# Autodesk Inventor assembly: 000 Ensamblaje_3d_Welding_Tooling - BASIC
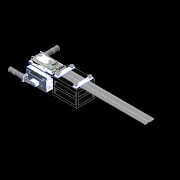
[picture p0: Inventor's stored thumbnail of the model, 180x180]
Saved by Autodesk Inventor 2018.3 (Build 223284000, 284)
## iProperties
Created: 2026-01-13
Part Number: 000 Ensamblaje_3d_Welding_Tooling - BASIC
Document SubType Name: Assembly
Designer: aca6
Mass: 2650.67 g
Surface Area: 3394.3 cm^2
Volume: 1053.59 cm^3
Density: 2.51584 g/cm^3
Manufacturer-1: {"Name": "Embention Sistemas Inteligentes S.A.", "PartNumber": "3d_Welding_Tooling - BASIC", "Link": ""}
Manufacturer-2: {"Name": "", "PartNumber": "", "Link": ""}
Manufacturer-3: {"Name": "", "PartNumber": "", "Link": ""}
Manufacturer-4: {"Name": "", "PartNumber": "", "Link": ""}
Manufacturer-5: {"Name": "", "PartNumber": "", "Link": ""}
Provider-1: {"Name": "", "PartNumber": "", "Link": ""}
Provider-2: {"Name": "", "PartNumber": "", "Link": ""}
Provider-3: {"Name": "", "PartNumber": "", "Link": ""}
Provider-4: {"Name": "", "PartNumber": "", "Link": ""}
Provider-5: {"Name": "", "PartNumber": "", "Link": ""}
Author: aca6
## Documents named in this file (29)
- C:\Users\aca6\git\LM\items\hw_LM\variants\items\Welding Tooling\3d\000 Ensamblaje_3d_Welding_Tooling - BASIC.iam
- C:\Users\aca6\git\LM\items\hw_LM\variants\items\Welding Tooling\3d\3d_Welding_Tooling - Adapter.ipt
- C:\Users\aca6\git\LM\items\hw_LM\variants\items\Welding Tooling\3d\3d_Welding_Tooling - Welding Placement.ipt
- C:\Users\aca6\git\LM\items\hw_LM\variants\items\Welding Tooling\3d\3d_Welding_Tooling -  Guide Pin.ipt
- C:\Users\aca6\git\LM\items\hw_LM\variants\items\Welding Tooling\3d\3d_Welding_Tooling - Wire.ipt
- C:\Users\aca6\git\LM\items\hw_LM\variants\items\Welding Tooling\3d\3d_Welding_Tooling - Bot Wire.ipt
- C:\Users\aca6\git\LM\items\hw_LM\variants\items\Welding Tooling\3d\3d_Welding_Tooling - Top Adapter.ipt
- C:\Users\aca6\git\LM\items\hw_LM\variants\items\Welding Tooling\3d\3d_Welding_Tooling - Moving base.ipt
- C:\Users\aca6\git\LM\items\hw_LM\variants\items\Welding Tooling\3d\3d_Welding_Tooling - Fixed base.ipt
- C:\Users\aca6\git\LM\items\hw_LM\variants\items\Welding Tooling\3d\3d_Welding_Tooling - Acetal Stick.ipt
- C:\Users\aca6\git\LM\items\hw_LM\variants\items\Welding Tooling\3d\3d_Welding_Tooling -  4x14 Guide Pin.ipt
- C:\Users\aca6\git\LM\items\hw_LM\variants\items\Welding Tooling\3d\3d_Welding_Tooling - Upper fixed base.ipt
- C:\Users\aca6\git\LM\items\hw_LM\variants\items\Welding Tooling\3d\3d_Welding_Tooling - Upper moving base.ipt
- C:\Users\aca6\git\LM\items\_accesories\Tornilleria\Tornillos\3d_DIN 7991\3d\A4 Black Inox\DIN 7991 - M3x14 Black INOX.ipt
- C:\Users\aca6\git\LM\items\_accesories\Tornilleria\Tornillos\3d_DIN 7991\3d\A4 Black Inox\DIN 7991 - M3x12 Black INOX.ipt
- C:\Users\aca6\git\LM\items\hw_LM\variants\items\Welding Tooling\3d\3d_Welding_Tooling -  Micrometer.ipt
- C:\Users\aca6\git\LM\items\hw_LM\variants\items\Welding Tooling\3d\3d_Welding_Tooling -  Micrometer Nut.ipt
- C:\Users\aca6\git\LM\items\hw_LM\variants\items\Welding Tooling\3d\3d_Welding_Tooling - Fixed Block.ipt
- C:\Users\aca6\git\LM\items\hw_LM\variants\items\Welding Tooling\3d\3d_Welding_Tooling -  Tab.ipt
- C:\Users\aca6\git\LM\items\hw_LM\variants\items\Welding Tooling\3d\3d_Welding_Tooling -  Moving Block.ipt
- C:\Users\aca6\git\LM\items\_accesories\Tornilleria\Tornillos\3d_Accu Group\3d\Prisionero nylon M4x7 REF SSN-M4-7.ipt
- C:\Users\aca6\git\LM\items\_accesories\Tornilleria\Tornillos\3d_DIN 912\3d\A4 Inox\DIN 912 - M3 x 0,5 x 8 -  INOX.ipt
- C:\Users\aca6\git\LM\items\_accesories\Tornilleria\Tornillos\3d_DIN 912\3d\A4 Inox\DIN 912 - M3 x 0,5 x 30 -  INOX.ipt
- C:\Users\aca6\git\LM\items\_accesories\Tornilleria\Tornillos\3d_DIN 912\3d\A4 Inox\DIN 912 - M3 x 0,5 x 10 -  INOX.ipt
- C:\Users\aca6\git\LM\items\_accesories\Tornilleria\Insertos\3d_Genéricos\3d\Inserto roscado M4x5.6x7.95.ipt
- C:\Users\aca6\git\LM\items\hw_LM\variants\items\Welding Tooling\3d\Knurled Screw_ Stainless Steel DIN 464-M4-10-A4.ipt
- C:\Users\aca6\git\LM\items\3d_LM\variants\BASIC\dummy\3d_LM - BASIC - welding tooling_dummy.ipt
- C:\Users\aca6\git\LM\items\3d_LM\3d\3d_LM - Bottom Wire - Phantom.ipt
- C:\Users\aca6\git\LM\items\3d_LM\3d\3d_LM - Top Wire - Phantom.ipt
## Components (69 placed, 28 different names)
1. 3d_Welding_Tooling - Adapter:1 — Flush:3, Mate:12, Mate:13, Mate:14, Mate:15, Mate:16, Mate:22, Mate:23, Mate:24, Flush:14, Mate:89, Mate:107, Flush:28, Flush:29, Mate:108, Mate:109, Mate:110, Mate:111, Tangent:5, Tangent:6, Tangent:7, Tangent:8, Flush:120
2. 3d_Welding_Tooling - Welding Placement:1 — Flush:3, Mate:89, Flush:120, Mate:126, Mate:127, Mate:128, Mate:129, Mate:130, Mate:131, Mate:136, Mate:137, Mate:204, Mate:205, Mate:206, Mate:207, Mate:208, Flush:141, Flush:142, Flush:143
3. 3d_Welding_Tooling -  Guide Pin:1 — Mate:12, Mate:16, Mate:23, Mate:50, Mate:238
4. 3d_Welding_Tooling -  Guide Pin:2 — Mate:13, Mate:15, Mate:22, Mate:49, Mate:239
5. 3d_Welding_Tooling -  Guide Pin:3 — Mate:14, Mate:24
6. 3d_Welding_Tooling - Top Adapter:1 — Flush:14, Mate:49, Mate:50, Mate:240
7. 3d_Welding_Tooling - Moving base:1 — Mate:58, Flush:18, Mate:59, Mate:60, Mate:94, Mate:95, Mate:96, Flush:123, Mate:173, Flush:140
8. 3d_Welding_Tooling - Fixed base:1 — Mate:58, Flush:18, Flush:19, Mate:61, Mate:62, Flush:20, Flush:123, Mate:163, Mate:165, Flush:124, Flush:125, Mate:168, Flush:129, Flush:130, Mate:178, Flush:135, Mate:179, Flush:136
9. 3d_Welding_Tooling - Acetal Stick:1 — Mate:59, Mate:60, Flush:19
10. 3d_Welding_Tooling - Acetal Stick:2 — Mate:61, Mate:62, Flush:20
11. 3d_Welding_Tooling -  4x14 Guide Pin:1 — Mate:128, Mate:129
12. 3d_Welding_Tooling -  4x14 Guide Pin:2 — Mate:126, Mate:127
13. 3d_Welding_Tooling - Upper fixed base:1 — Mate:94, Mate:95, Mate:96, Mate:97, Mate:98, Mate:99, Mate:100, Flush:26, Flush:27, Mate:101, Mate:103, Mate:104, Mate:105, Mate:106, Tangent:1, Tangent:2, Tangent:3, Tangent:4, Mate:158, Flush:121, Flush:122, Mate:162, Mate:164, Flush:126, Flush:127, Flush:128, Mate:180, Flush:137, Mate:181, Flush:138
14. 3d_Welding_Tooling - Acetal Stick:3 — Mate:97, Mate:98, Flush:27
15. 3d_Welding_Tooling - Acetal Stick:4 — Mate:99, Mate:100, Flush:26, Mate:102
16. 3d_Welding_Tooling - Upper moving base:1 — Mate:101, Mate:102, Mate:107, Flush:28, Flush:29, Mate:160, Flush:122, Mate:174, Mate:175, Mate:176, Mate:177, Flush:131, Flush:132, Flush:133, Flush:134, Flush:139
17. DIN 7991 - M3x14 Black INOX:1 — Mate:105, Tangent:3
18. DIN 7991 - M3x14 Black INOX:2 — Mate:106, Tangent:2
19. DIN 7991 - M3x14 Black INOX:3 — Mate:103, Tangent:4
20. DIN 7991 - M3x14 Black INOX:4 — Mate:104, Tangent:1
21. DIN 7991 - M3x12 Black INOX:1 — Mate:109, Tangent:8
22. DIN 7991 - M3x12 Black INOX:2 — Mate:111, Tangent:6
23. DIN 7991 - M3x12 Black INOX:3 — Mate:110, Tangent:5
24. DIN 7991 - M3x12 Black INOX:4 — Mate:108, Tangent:7
25. 3d_Welding_Tooling -  Micrometer Nut:1 — Mate:171, Mate:172
26. 3d_Welding_Tooling -  Tab:1 — Mate:130, Mate:131, Mate:217, Mate:223
27. 3d_Welding_Tooling -  Tab:2 — Mate:136, Mate:137, Mate:219, Mate:221
28. 3d_Welding_Tooling -  Micrometer:2 — Mate:187
29. 3d_Welding_Tooling -  Micrometer Nut:2
30. 3d_Welding_Tooling - Fixed Block:2 — Mate:158, Flush:121, Flush:128, Mate:196, Mate:197, Mate:198, Mate:199
31. 3d_Welding_Tooling -  Moving Block:1 — Mate:160, Mate:184, Mate:185, Mate:187, Flush:139, Mate:192, Mate:193, Mate:194, Mate:195
32. Prisionero nylon M4x7 REF SSN-M4-7:1 — Mate:162, Flush:126
33. Prisionero nylon M4x7 REF SSN-M4-7:2 — Mate:163, Flush:125
34. Prisionero nylon M4x7 REF SSN-M4-7:3 — Mate:165, Flush:124
35. Prisionero nylon M4x7 REF SSN-M4-7:4 — Mate:164, Flush:127
36. 3d_Welding_Tooling - Fixed Block:3 — Mate:168, Flush:129, Flush:130, Mate:169, Mate:170, Mate:172, Mate:200, Mate:201, Mate:202, Mate:203
37. 3d_Welding_Tooling -  Micrometer:3 — Mate:169, Mate:170, Mate:171, Mate:186
38. 3d_Welding_Tooling -  Moving Block:2 — Mate:173, Mate:182, Mate:183, Mate:186, Flush:140, Mate:188, Mate:189, Mate:190, Mate:191
39. Prisionero nylon M4x7 REF SSN-M4-7:5 — Mate:174, Flush:132
40. Prisionero nylon M4x7 REF SSN-M4-7:6 — Mate:177, Flush:131
41. Prisionero nylon M4x7 REF SSN-M4-7:7 — Mate:176, Flush:133
42. Prisionero nylon M4x7 REF SSN-M4-7:8 — Mate:175, Flush:134
43. Prisionero nylon M4x7 REF SSN-M4-7:9 — Mate:178, Flush:135
44. Prisionero nylon M4x7 REF SSN-M4-7:10 — Mate:179, Flush:136
45. Prisionero nylon M4x7 REF SSN-M4-7:11 — Mate:180, Flush:137
46. Prisionero nylon M4x7 REF SSN-M4-7:12 — Mate:181, Flush:138
47. DIN 912 - M3 x 0,5 x 8 -  INOX:1 — Mate:184, Mate:185
48. DIN 912 - M3 x 0,5 x 8 -  INOX:2 — Mate:182, Mate:183
49. DIN 912 - M3 x 0,5 x 30 -  INOX:4 — Mate:189, Mate:191
50. DIN 912 - M3 x 0,5 x 30 -  INOX:3 — Mate:188, Mate:190
51. DIN 912 - M3 x 0,5 x 30 -  INOX:1 — Mate:192, Mate:195
52. DIN 912 - M3 x 0,5 x 30 -  INOX:2 — Mate:193, Mate:194
53. DIN 912 - M3 x 0,5 x 10 -  INOX:1 — Mate:197, Mate:198
54. DIN 912 - M3 x 0,5 x 10 -  INOX:2 — Mate:196, Mate:199
55. DIN 912 - M3 x 0,5 x 10 -  INOX:3 — Mate:201, Mate:202
56. DIN 912 - M3 x 0,5 x 10 -  INOX:4 — Mate:200, Mate:203
57. Inserto roscado M4x5.6x7.95:1 — Mate:204, Mate:205, Mate:216
58. Inserto roscado M4x5.6x7.95:2 — Mate:207, Flush:143, Mate:218
59. Inserto roscado M4x5.6x7.95:3 — Mate:208, Flush:142, Mate:220
60. Inserto roscado M4x5.6x7.95:4 — Mate:206, Flush:141, Mate:222
61. Knurled Screw_ Stainless Steel DIN 464-M4-10-A4:1 — Mate:216, Mate:217
62. Knurled Screw_ Stainless Steel DIN 464-M4-10-A4:2 — Mate:222, Mate:223
63. Knurled Screw_ Stainless Steel DIN 464-M4-10-A4:3 — Mate:220, Mate:221
64. Knurled Screw_ Stainless Steel DIN 464-M4-10-A4:4 — Mate:218, Mate:219
65. 3d_LM - Top Wire - Phantom:1 — Mate:244, Mate:245, Mate:246, Mate:250, Mate:251, Mate:252
66. 3d_LM - Bottom Wire - Phantom:1 — Mate:241, Mate:242, Mate:243, Mate:247, Mate:248, Mate:249
67. 3d_LM - BASIC - welding tooling_dummy:1 — Mate:238, Mate:239, Mate:240, Mate:247, Mate:248, Mate:249, Mate:250, Mate:251, Mate:252
68. 3d_Welding_Tooling - Wire:1 — Mate:244, Mate:245, Mate:246
69. 3d_Welding_Tooling - Bot Wire:1 — Mate:241, Mate:242, Mate:243
## Relationships (157: Mate 116, Flush 33, Tangent 8)
- Flush:3 (-60 mm): 3d_Welding_Tooling - Adapter:1 ↔ 3d_Welding_Tooling - Welding Placement:1
- Mate:12: 3d_Welding_Tooling - Adapter:1 ↔ 3d_Welding_Tooling -  Guide Pin:1
- Mate:13: 3d_Welding_Tooling - Adapter:1 ↔ 3d_Welding_Tooling -  Guide Pin:2
- Mate:14: 3d_Welding_Tooling - Adapter:1 ↔ 3d_Welding_Tooling -  Guide Pin:3
- Mate:15: 3d_Welding_Tooling - Adapter:1 ↔ 3d_Welding_Tooling -  Guide Pin:2
- Mate:16: 3d_Welding_Tooling - Adapter:1 ↔ 3d_Welding_Tooling -  Guide Pin:1
- Mate:22: 3d_Welding_Tooling - Adapter:1 ↔ 3d_Welding_Tooling -  Guide Pin:2
- Mate:23: 3d_Welding_Tooling - Adapter:1 ↔ 3d_Welding_Tooling -  Guide Pin:1
- Mate:24: 3d_Welding_Tooling - Adapter:1 ↔ 3d_Welding_Tooling -  Guide Pin:3
- Flush:14: 3d_Welding_Tooling - Adapter:1 ↔ 3d_Welding_Tooling - Top Adapter:1
- Mate:49: 3d_Welding_Tooling -  Guide Pin:2 ↔ 3d_Welding_Tooling - Top Adapter:1
- Mate:50: 3d_Welding_Tooling -  Guide Pin:1 ↔ 3d_Welding_Tooling - Top Adapter:1
- Mate:58: 3d_Welding_Tooling - Moving base:1 ↔ 3d_Welding_Tooling - Fixed base:1
- Flush:18: 3d_Welding_Tooling - Moving base:1 ↔ 3d_Welding_Tooling - Fixed base:1
- Mate:59: 3d_Welding_Tooling - Moving base:1 ↔ 3d_Welding_Tooling - Acetal Stick:1
- Mate:60: 3d_Welding_Tooling - Moving base:1 ↔ 3d_Welding_Tooling - Acetal Stick:1
- Mate:61: 3d_Welding_Tooling - Fixed base:1 ↔ 3d_Welding_Tooling - Acetal Stick:2
- Mate:62: 3d_Welding_Tooling - Fixed base:1 ↔ 3d_Welding_Tooling - Acetal Stick:2
- Flush:19: 3d_Welding_Tooling - Fixed base:1 ↔ 3d_Welding_Tooling - Acetal Stick:1
- Flush:20: 3d_Welding_Tooling - Fixed base:1 ↔ 3d_Welding_Tooling - Acetal Stick:2
- Mate:89 (3 mm): 3d_Welding_Tooling - Adapter:1 ↔ 3d_Welding_Tooling - Welding Placement:1
- Mate:94: 3d_Welding_Tooling - Moving base:1 ↔ 3d_Welding_Tooling - Upper fixed base:1
- Mate:95: 3d_Welding_Tooling - Moving base:1 ↔ 3d_Welding_Tooling - Upper fixed base:1
- Mate:96: 3d_Welding_Tooling - Moving base:1 ↔ 3d_Welding_Tooling - Upper fixed base:1
- Mate:97: 3d_Welding_Tooling - Upper fixed base:1 ↔ 3d_Welding_Tooling - Acetal Stick:3
- Mate:98: 3d_Welding_Tooling - Upper fixed base:1 ↔ 3d_Welding_Tooling - Acetal Stick:3
- Mate:99: 3d_Welding_Tooling - Upper fixed base:1 ↔ 3d_Welding_Tooling - Acetal Stick:4
- Mate:100: 3d_Welding_Tooling - Upper fixed base:1 ↔ 3d_Welding_Tooling - Acetal Stick:4
- Flush:26: 3d_Welding_Tooling - Upper fixed base:1 ↔ 3d_Welding_Tooling - Acetal Stick:4
- Flush:27: 3d_Welding_Tooling - Upper fixed base:1 ↔ 3d_Welding_Tooling - Acetal Stick:3
- Mate:101: 3d_Welding_Tooling - Upper fixed base:1 ↔ 3d_Welding_Tooling - Upper moving base:1
- Mate:102: 3d_Welding_Tooling - Acetal Stick:4 ↔ 3d_Welding_Tooling - Upper moving base:1
- Mate:103: 3d_Welding_Tooling - Upper fixed base:1 ↔ DIN 7991 - M3x14 Black INOX:3
- Mate:104: 3d_Welding_Tooling - Upper fixed base:1 ↔ DIN 7991 - M3x14 Black INOX:4
- Mate:105: 3d_Welding_Tooling - Upper fixed base:1 ↔ DIN 7991 - M3x14 Black INOX:1
- Mate:106: 3d_Welding_Tooling - Upper fixed base:1 ↔ DIN 7991 - M3x14 Black INOX:2
- Tangent:1: 3d_Welding_Tooling - Upper fixed base:1 ↔ DIN 7991 - M3x14 Black INOX:4
- Tangent:2: 3d_Welding_Tooling - Upper fixed base:1 ↔ DIN 7991 - M3x14 Black INOX:2
- Tangent:3: 3d_Welding_Tooling - Upper fixed base:1 ↔ DIN 7991 - M3x14 Black INOX:1
- Tangent:4: 3d_Welding_Tooling - Upper fixed base:1 ↔ DIN 7991 - M3x14 Black INOX:3
- Mate:107: 3d_Welding_Tooling - Adapter:1 ↔ 3d_Welding_Tooling - Upper moving base:1
- Flush:28 (18.75 mm): 3d_Welding_Tooling - Adapter:1 ↔ 3d_Welding_Tooling - Upper moving base:1
- Flush:29 (-9.684 mm): 3d_Welding_Tooling - Adapter:1 ↔ 3d_Welding_Tooling - Upper moving base:1
- Mate:108: 3d_Welding_Tooling - Adapter:1 ↔ DIN 7991 - M3x12 Black INOX:4
- Mate:109: 3d_Welding_Tooling - Adapter:1 ↔ DIN 7991 - M3x12 Black INOX:1
- Mate:110: 3d_Welding_Tooling - Adapter:1 ↔ DIN 7991 - M3x12 Black INOX:3
- Mate:111: 3d_Welding_Tooling - Adapter:1 ↔ DIN 7991 - M3x12 Black INOX:2
- Tangent:5: 3d_Welding_Tooling - Adapter:1 ↔ DIN 7991 - M3x12 Black INOX:3
- Tangent:6: 3d_Welding_Tooling - Adapter:1 ↔ DIN 7991 - M3x12 Black INOX:2
- Tangent:7: 3d_Welding_Tooling - Adapter:1 ↔ DIN 7991 - M3x12 Black INOX:4
- Tangent:8: 3d_Welding_Tooling - Adapter:1 ↔ DIN 7991 - M3x12 Black INOX:1
- Flush:120 (-13.75 mm): 3d_Welding_Tooling - Adapter:1 ↔ 3d_Welding_Tooling - Welding Placement:1
- Mate:126: 3d_Welding_Tooling - Welding Placement:1 ↔ 3d_Welding_Tooling -  4x14 Guide Pin:2
- Mate:127: 3d_Welding_Tooling - Welding Placement:1 ↔ 3d_Welding_Tooling -  4x14 Guide Pin:2
- Mate:128: 3d_Welding_Tooling - Welding Placement:1 ↔ 3d_Welding_Tooling -  4x14 Guide Pin:1
- Mate:129: 3d_Welding_Tooling - Welding Placement:1 ↔ 3d_Welding_Tooling -  4x14 Guide Pin:1
- Mate:130 (2.5 mm): 3d_Welding_Tooling - Welding Placement:1 ↔ 3d_Welding_Tooling -  Tab:1
- Mate:131: 3d_Welding_Tooling - Welding Placement:1 ↔ 3d_Welding_Tooling -  Tab:1
- Mate:136: 3d_Welding_Tooling - Welding Placement:1 ↔ 3d_Welding_Tooling -  Tab:2
- Mate:137 (2.5 mm): 3d_Welding_Tooling - Welding Placement:1 ↔ 3d_Welding_Tooling -  Tab:2
- [Mate]: 3d_Welding_Tooling -  Micrometer:2 ↔ 3d_Welding_Tooling - Fixed Block:2
- [Mate]: 3d_Welding_Tooling -  Micrometer:2 ↔ 3d_Welding_Tooling - Fixed Block:2
- [Mate]: 3d_Welding_Tooling -  Micrometer:2 ↔ 3d_Welding_Tooling -  Micrometer Nut:2
- [Mate]: 3d_Welding_Tooling -  Micrometer Nut:2 ↔ 3d_Welding_Tooling - Fixed Block:2
- Mate:158: 3d_Welding_Tooling - Upper fixed base:1 ↔ 3d_Welding_Tooling - Fixed Block:2
- Flush:121: 3d_Welding_Tooling - Upper fixed base:1 ↔ 3d_Welding_Tooling - Fixed Block:2
- Mate:160: 3d_Welding_Tooling - Upper moving base:1 ↔ 3d_Welding_Tooling -  Moving Block:1
- Flush:122: 3d_Welding_Tooling - Upper fixed base:1 ↔ 3d_Welding_Tooling - Upper moving base:1
- Flush:123: 3d_Welding_Tooling - Moving base:1 ↔ 3d_Welding_Tooling - Fixed base:1
- Mate:162: 3d_Welding_Tooling - Upper fixed base:1 ↔ Prisionero nylon M4x7 REF SSN-M4-7:1
- Mate:163: 3d_Welding_Tooling - Fixed base:1 ↔ Prisionero nylon M4x7 REF SSN-M4-7:2
- Mate:164: 3d_Welding_Tooling - Upper fixed base:1 ↔ Prisionero nylon M4x7 REF SSN-M4-7:4
- Mate:165: 3d_Welding_Tooling - Fixed base:1 ↔ Prisionero nylon M4x7 REF SSN-M4-7:3
- Flush:124: 3d_Welding_Tooling - Fixed base:1 ↔ Prisionero nylon M4x7 REF SSN-M4-7:3
- Flush:125: 3d_Welding_Tooling - Fixed base:1 ↔ Prisionero nylon M4x7 REF SSN-M4-7:2
- Flush:126: 3d_Welding_Tooling - Upper fixed base:1 ↔ Prisionero nylon M4x7 REF SSN-M4-7:1
- Flush:127: 3d_Welding_Tooling - Upper fixed base:1 ↔ Prisionero nylon M4x7 REF SSN-M4-7:4
- Flush:128: 3d_Welding_Tooling - Upper fixed base:1 ↔ 3d_Welding_Tooling - Fixed Block:2
- Mate:168: 3d_Welding_Tooling - Fixed base:1 ↔ 3d_Welding_Tooling - Fixed Block:3
- Flush:129: 3d_Welding_Tooling - Fixed base:1 ↔ 3d_Welding_Tooling - Fixed Block:3
- Flush:130: 3d_Welding_Tooling - Fixed base:1 ↔ 3d_Welding_Tooling - Fixed Block:3
- Mate:169: 3d_Welding_Tooling - Fixed Block:3 ↔ 3d_Welding_Tooling -  Micrometer:3
- Mate:170: 3d_Welding_Tooling - Fixed Block:3 ↔ 3d_Welding_Tooling -  Micrometer:3
- Mate:171: 3d_Welding_Tooling -  Micrometer Nut:1 ↔ 3d_Welding_Tooling -  Micrometer:3
- Mate:172: 3d_Welding_Tooling -  Micrometer Nut:1 ↔ 3d_Welding_Tooling - Fixed Block:3
- Mate:173: 3d_Welding_Tooling - Moving base:1 ↔ 3d_Welding_Tooling -  Moving Block:2
- Mate:174: 3d_Welding_Tooling - Upper moving base:1 ↔ Prisionero nylon M4x7 REF SSN-M4-7:5
- Mate:175: 3d_Welding_Tooling - Upper moving base:1 ↔ Prisionero nylon M4x7 REF SSN-M4-7:8
- Mate:176: 3d_Welding_Tooling - Upper moving base:1 ↔ Prisionero nylon M4x7 REF SSN-M4-7:7
- Mate:177: 3d_Welding_Tooling - Upper moving base:1 ↔ Prisionero nylon M4x7 REF SSN-M4-7:6
- Flush:131: 3d_Welding_Tooling - Upper moving base:1 ↔ Prisionero nylon M4x7 REF SSN-M4-7:6
- Flush:132: 3d_Welding_Tooling - Upper moving base:1 ↔ Prisionero nylon M4x7 REF SSN-M4-7:5
- Flush:133: 3d_Welding_Tooling - Upper moving base:1 ↔ Prisionero nylon M4x7 REF SSN-M4-7:7
- Flush:134: 3d_Welding_Tooling - Upper moving base:1 ↔ Prisionero nylon M4x7 REF SSN-M4-7:8
- Mate:178: 3d_Welding_Tooling - Fixed base:1 ↔ Prisionero nylon M4x7 REF SSN-M4-7:9
- Flush:135: 3d_Welding_Tooling - Fixed base:1 ↔ Prisionero nylon M4x7 REF SSN-M4-7:9
- Mate:179: 3d_Welding_Tooling - Fixed base:1 ↔ Prisionero nylon M4x7 REF SSN-M4-7:10
- Flush:136: 3d_Welding_Tooling - Fixed base:1 ↔ Prisionero nylon M4x7 REF SSN-M4-7:10
- Mate:180: 3d_Welding_Tooling - Upper fixed base:1 ↔ Prisionero nylon M4x7 REF SSN-M4-7:11
- Flush:137: 3d_Welding_Tooling - Upper fixed base:1 ↔ Prisionero nylon M4x7 REF SSN-M4-7:11
- Mate:181: 3d_Welding_Tooling - Upper fixed base:1 ↔ Prisionero nylon M4x7 REF SSN-M4-7:12
- Flush:138: 3d_Welding_Tooling - Upper fixed base:1 ↔ Prisionero nylon M4x7 REF SSN-M4-7:12
- Mate:182: 3d_Welding_Tooling -  Moving Block:2 ↔ DIN 912 - M3 x 0,5 x 8 -  INOX:2
- Mate:183: 3d_Welding_Tooling -  Moving Block:2 ↔ DIN 912 - M3 x 0,5 x 8 -  INOX:2
- Mate:184: 3d_Welding_Tooling -  Moving Block:1 ↔ DIN 912 - M3 x 0,5 x 8 -  INOX:1
- Mate:185: 3d_Welding_Tooling -  Moving Block:1 ↔ DIN 912 - M3 x 0,5 x 8 -  INOX:1
- Mate:186: 3d_Welding_Tooling -  Micrometer:3 ↔ 3d_Welding_Tooling -  Moving Block:2
- Mate:187: 3d_Welding_Tooling -  Micrometer:2 ↔ 3d_Welding_Tooling -  Moving Block:1
- Flush:139 (50 mm): 3d_Welding_Tooling - Upper moving base:1 ↔ 3d_Welding_Tooling -  Moving Block:1
- Flush:140 (50 mm): 3d_Welding_Tooling - Moving base:1 ↔ 3d_Welding_Tooling -  Moving Block:2
- Mate:188: 3d_Welding_Tooling -  Moving Block:2 ↔ DIN 912 - M3 x 0,5 x 30 -  INOX:3
- Mate:189: 3d_Welding_Tooling -  Moving Block:2 ↔ DIN 912 - M3 x 0,5 x 30 -  INOX:4
- Mate:190: 3d_Welding_Tooling -  Moving Block:2 ↔ DIN 912 - M3 x 0,5 x 30 -  INOX:3
- Mate:191: 3d_Welding_Tooling -  Moving Block:2 ↔ DIN 912 - M3 x 0,5 x 30 -  INOX:4
- Mate:192: 3d_Welding_Tooling -  Moving Block:1 ↔ DIN 912 - M3 x 0,5 x 30 -  INOX:1
- Mate:193: 3d_Welding_Tooling -  Moving Block:1 ↔ DIN 912 - M3 x 0,5 x 30 -  INOX:2
- Mate:194: 3d_Welding_Tooling -  Moving Block:1 ↔ DIN 912 - M3 x 0,5 x 30 -  INOX:2
- Mate:195: 3d_Welding_Tooling -  Moving Block:1 ↔ DIN 912 - M3 x 0,5 x 30 -  INOX:1
- Mate:196: 3d_Welding_Tooling - Fixed Block:2 ↔ DIN 912 - M3 x 0,5 x 10 -  INOX:2
- Mate:197: 3d_Welding_Tooling - Fixed Block:2 ↔ DIN 912 - M3 x 0,5 x 10 -  INOX:1
- Mate:198: 3d_Welding_Tooling - Fixed Block:2 ↔ DIN 912 - M3 x 0,5 x 10 -  INOX:1
- Mate:199: 3d_Welding_Tooling - Fixed Block:2 ↔ DIN 912 - M3 x 0,5 x 10 -  INOX:2
- Mate:200: 3d_Welding_Tooling - Fixed Block:3 ↔ DIN 912 - M3 x 0,5 x 10 -  INOX:4
- Mate:201: 3d_Welding_Tooling - Fixed Block:3 ↔ DIN 912 - M3 x 0,5 x 10 -  INOX:3
- Mate:202: 3d_Welding_Tooling - Fixed Block:3 ↔ DIN 912 - M3 x 0,5 x 10 -  INOX:3
- Mate:203: 3d_Welding_Tooling - Fixed Block:3 ↔ DIN 912 - M3 x 0,5 x 10 -  INOX:4
- Mate:204: 3d_Welding_Tooling - Welding Placement:1 ↔ Inserto roscado M4x5.6x7.95:1
- Mate:205: 3d_Welding_Tooling - Welding Placement:1 ↔ Inserto roscado M4x5.6x7.95:1
- Mate:206: 3d_Welding_Tooling - Welding Placement:1 ↔ Inserto roscado M4x5.6x7.95:4
- Mate:207: 3d_Welding_Tooling - Welding Placement:1 ↔ Inserto roscado M4x5.6x7.95:2
- Mate:208: 3d_Welding_Tooling - Welding Placement:1 ↔ Inserto roscado M4x5.6x7.95:3
- Flush:141: 3d_Welding_Tooling - Welding Placement:1 ↔ Inserto roscado M4x5.6x7.95:4
- Flush:142: 3d_Welding_Tooling - Welding Placement:1 ↔ Inserto roscado M4x5.6x7.95:3
- Flush:143: 3d_Welding_Tooling - Welding Placement:1 ↔ Inserto roscado M4x5.6x7.95:2
- Mate:216: Inserto roscado M4x5.6x7.95:1 ↔ Knurled Screw_ Stainless Steel DIN 464-M4-10-A4:1
- Mate:217: 3d_Welding_Tooling -  Tab:1 ↔ Knurled Screw_ Stainless Steel DIN 464-M4-10-A4:1
- Mate:218: Inserto roscado M4x5.6x7.95:2 ↔ Knurled Screw_ Stainless Steel DIN 464-M4-10-A4:4
- Mate:219: 3d_Welding_Tooling -  Tab:2 ↔ Knurled Screw_ Stainless Steel DIN 464-M4-10-A4:4
- Mate:220: Inserto roscado M4x5.6x7.95:3 ↔ Knurled Screw_ Stainless Steel DIN 464-M4-10-A4:3
- Mate:221: 3d_Welding_Tooling -  Tab:2 ↔ Knurled Screw_ Stainless Steel DIN 464-M4-10-A4:3
- Mate:222: Inserto roscado M4x5.6x7.95:4 ↔ Knurled Screw_ Stainless Steel DIN 464-M4-10-A4:2
- Mate:223: 3d_Welding_Tooling -  Tab:1 ↔ Knurled Screw_ Stainless Steel DIN 464-M4-10-A4:2
- Mate:238: 3d_Welding_Tooling -  Guide Pin:1 ↔ 3d_LM - BASIC - welding tooling_dummy:1
- Mate:239: 3d_Welding_Tooling -  Guide Pin:2 ↔ 3d_LM - BASIC - welding tooling_dummy:1
- Mate:240: 3d_Welding_Tooling - Top Adapter:1 ↔ 3d_LM - BASIC - welding tooling_dummy:1
- Mate:241: 3d_LM - Bottom Wire - Phantom:1 ↔ 3d_Welding_Tooling - Bot Wire:1
- Mate:242: 3d_LM - Bottom Wire - Phantom:1 ↔ 3d_Welding_Tooling - Bot Wire:1
- Mate:243: 3d_LM - Bottom Wire - Phantom:1 ↔ 3d_Welding_Tooling - Bot Wire:1
- Mate:244: 3d_LM - Top Wire - Phantom:1 ↔ 3d_Welding_Tooling - Wire:1
- Mate:245: 3d_LM - Top Wire - Phantom:1 ↔ 3d_Welding_Tooling - Wire:1
- Mate:246: 3d_LM - Top Wire - Phantom:1 ↔ 3d_Welding_Tooling - Wire:1
- Mate:247: 3d_LM - Bottom Wire - Phantom:1 ↔ 3d_LM - BASIC - welding tooling_dummy:1
- Mate:248: 3d_LM - Bottom Wire - Phantom:1 ↔ 3d_LM - BASIC - welding tooling_dummy:1
- Mate:249 (-7 mm): 3d_LM - Bottom Wire - Phantom:1 ↔ 3d_LM - BASIC - welding tooling_dummy:1
- Mate:250: 3d_LM - Top Wire - Phantom:1 ↔ 3d_LM - BASIC - welding tooling_dummy:1
- Mate:251: 3d_LM - Top Wire - Phantom:1 ↔ 3d_LM - BASIC - welding tooling_dummy:1
- Mate:252 (-7 mm): 3d_LM - Top Wire - Phantom:1 ↔ 3d_LM - BASIC - welding tooling_dummy:1
## Named parameters: d236_d199 = 0 mm, d237_d201 = 0 mm, d238_d203 = 0 mm, d239_d204 = 0 mm
